# Autodesk Inventor assembly: SHOT_1_002_ShooterAssembly
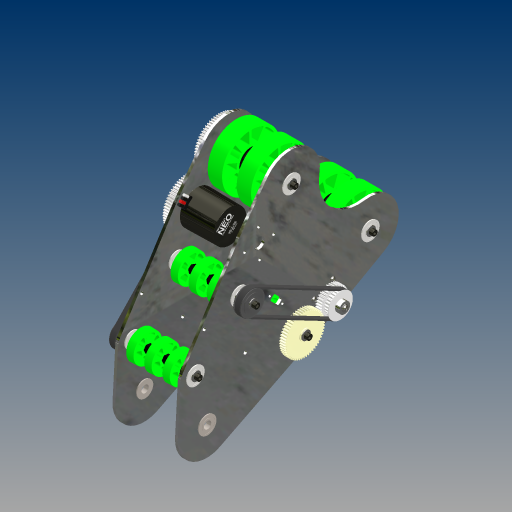
[picture p0: Inventor's stored thumbnail of the model, 512x512]
Saved by Autodesk Inventor 2024.3 (Build 283343000, 343)
## iProperties
Created: 2024-08-07
Part Number: SHOT_1_002_ShooterAssembly
Document SubType Name: Assembly
Designer: Kenji
Mass: 1474.99 g
Surface Area: 3908.93 cm^2
Volume: 710.058 cm^3
Density: 2.07728 g/cm^3
Author: Kenji
## Documents named in this file (27)
- C:\Users\Kenji\Documents\GitHub\1622-2024-Summer-CAD-A-Thon\Shooter\SHOT_1_002_ShooterAssembly.iam
- C:\Users\Kenji\Documents\GitHub\1622-2024-Summer-CAD-A-Thon\Shooter\SHOT_1_001_ShooterPlate.ipt
- C:\Users\Kenji\Documents\GitHub\1622-2024-Summer-CAD-A-Thon\COTS Library\Motion\Wheels\Compliant Wheels\4in compliant wheels\0.500in hex bore\COTS_am-3462_4indiameter_0.500inhexbore_durometer35A_CompliantWheel.ipt
- C:\Users\Kenji\Documents\GitHub\1622-2024-Summer-CAD-A-Thon\COTS Library\Motion\Bearings\COTS_WCP-0783_1.125ODHexBearing.ipt
- C:\Users\Kenji\Documents\GitHub\1622-2024-Summer-CAD-A-Thon\COTS Library\Motion\Bearings\COTS_WCP-0781_0.5ODCircularFlangedBearing.ipt
- C:\Users\Kenji\Documents\GitHub\1622-2024-Summer-CAD-A-Thon\COTS Library\Motors\COTS_REV-21-1650-V1.1_Neo1.1.ipt
- C:\Users\Kenji\Documents\GitHub\1622-2024-Summer-CAD-A-Thon\COTS Library\Motion\Wheels\Compliant Wheels\2in compliant wheels\0.500in hex bore\COTS_am-3462_2indiameter_0.500inhexbore_durometer35A_CompliantWheel.ipt
- C:\Users\Kenji\Documents\GitHub\1622-2024-Summer-CAD-A-Thon\COTS Library\Fasteners\Bolts\Button-Head\10-32\COTS_92949A265_1-2in long Stainless Steel Button Head Screw.ipt
- C:\Users\Kenji\Documents\GitHub\1622-2024-Summer-CAD-A-Thon\COTS Library\Motion\Pulleys\HTD5M\10mm Wide\COTS_HTD5M10mm24T_WCP-0564.ipt
- C:\Users\Kenji\Documents\GitHub\1622-2024-Summer-CAD-A-Thon\COTS Library\Adapters\COTS_REV-21-1879_8mmKeyTo0.5Hex.ipt
- C:\Users\Kenji\Documents\GitHub\1622-2024-Summer-CAD-A-Thon\COTS Library\Motion\Gears\20DP gears\Aluminum\COTS_WCP-0171_66T.ipt
- C:\Users\Kenji\Documents\GitHub\1622-2024-Summer-CAD-A-Thon\Shooter\SHOT_1_004_66TGear-24TPulley.ipt
- C:\Users\Kenji\Documents\GitHub\1622-2024-Summer-CAD-A-Thon\COTS Library\Motion\Gears\20DP gears\Aluminum\COTS_WCP-0717_54T.ipt
- C:\Users\Kenji\Documents\GitHub\1622-2024-Summer-CAD-A-Thon\Shooter\SHOT_1_005_36TGear-24TPulley.ipt
- C:\Users\Kenji\Documents\GitHub\1622-2024-Summer-CAD-A-Thon\Shooter\SHOT_1_014_Belt3.ipt
- C:\Users\Kenji\Documents\GitHub\1622-2024-Summer-CAD-A-Thon\Shooter\SHOT_1_013_Belt2.ipt
- C:\Users\Kenji\Documents\GitHub\1622-2024-Summer-CAD-A-Thon\Shooter\SHOT_1_012_Belt1.ipt
- C:\Users\Kenji\Documents\GitHub\1622-2024-Summer-CAD-A-Thon\Shooter\SHOT_1_010_Spacer1.ipt
- C:\Users\Kenji\Documents\GitHub\1622-2024-Summer-CAD-A-Thon\Shooter\SHOT_1_011_Spacer2.ipt
- C:\Users\Kenji\Documents\GitHub\1622-2024-Summer-CAD-A-Thon\Shooter\SHOT_1_006_HexShaft1.ipt
- C:\Users\Kenji\Documents\GitHub\1622-2024-Summer-CAD-A-Thon\Shooter\SHOT_1_007_HexShaft2.ipt
- C:\Users\Kenji\Documents\GitHub\1622-2024-Summer-CAD-A-Thon\Shooter\SHOT_1_008_HexShaft3.ipt
- C:\Users\Kenji\Documents\GitHub\1622-2024-Summer-CAD-A-Thon\Shooter\SHOT_1_009_HexShaft4.ipt
- C:\Users\Kenji\Documents\GitHub\1622-2024-Summer-CAD-A-Thon\COTS Library\Fasteners\Bolts\Socket-Head\0.25-20\COTS_91251A539_Black-Oxide Alloy Steel Socket Head Screw (1).ipt
- C:\Users\Kenji\Documents\GitHub\1622-2024-Summer-CAD-A-Thon\COTS Library\Fasteners\Washers\COTS_90107A029_316 Stainless Steel Washer.ipt
- C:\Users\Kenji\Documents\GitHub\1622-2024-Summer-CAD-A-Thon\COTS Library\Fasteners\Bolts\Button-Head\10-32\COTS_92949A267_18-8 Stainless Steel Button Head Hex Drive Screw (1).ipt
- C:\Users\Kenji\Documents\GitHub\1622-2024-Summer-CAD-A-Thon\COTS Library\Fasteners\Washers\COTS_91860A047_Size10Washer.ipt
## Components (83 placed, 26 different names)
1. SHOT_1_001_ShooterPlate:1 — Mate:140, Mate:141, Mate:142, Mate:143, Mate:144, Mate:148, Mate:150, Mate:151, Mate:152, Mate:153, Mate:155, Mate:160, Mate:161, Mate:163, Mate:164, Mate:165, Mate:166, Mate:167, Mate:168, Mate:169, Mate:170, Mate:171, Mate:172
2. SHOT_1_001_ShooterPlate:2 — Mate:140, Mate:141, Mate:145, Mate:147, Mate:149, Mate:156, Mate:157, Mate:158, Mate:159, Mate:173, Mate:174, Mate:175, Mate:176, Mate:177, Mate:178, Mate:179, Mate:180, Mate:181, Mate:183, Mate:192
3. COTS_WCP-0783_1.125ODHexBearing:1 — Mate:139, Flush:5, Mate:156, Mate:184, Mate:246
4. COTS_WCP-0783_1.125ODHexBearing:2 — Mate:146, Mate:147, Mate:149, Mate:193
5. COTS_WCP-0783_1.125ODHexBearing:3 — Mate:36, Mate:102, Flush:5, Mate:251
6. COTS_WCP-0783_1.125ODHexBearing:5 — Mate:50, Mate:136, Mate:155, Mate:244
7. COTS_WCP-0783_1.125ODHexBearing:9 — Mate:102, Flush:4, Mate:150, Mate:152, Mate:186, Mate:187
8. COTS_WCP-0783_1.125ODHexBearing:10 — Mate:31, Mate:104, Flush:4, Mate:151, Mate:188, Mate:213
9. COTS_WCP-0783_1.125ODHexBearing:11 — Mate:49, Mate:52, Mate:143, Mate:144, Mate:196, Mate:197
10. COTS_WCP-0783_1.125ODHexBearing:12 — Mate:154, Mate:157, Mate:189, Mate:190
11. COTS_WCP-0781_0.5ODCircularFlangedBearing:1 — Mate:138, Mate:158, Mate:159
12. COTS_WCP-0781_0.5ODCircularFlangedBearing:2 — Mate:138, Mate:160
13. COTS_REV-21-1650-V1.1_Neo1.1:1 — Mate:133, Mate:161, Mate:163, Mate:185, Mate:256, Mate:260, Mate:261, Mate:266
14. COTS_92949A265_1-2in long Stainless Steel Button Head Screw:1 — Mate:165, Mate:168, Mate:185
15. COTS_92949A265_1-2in long Stainless Steel Button Head Screw:2 — Mate:167, Mate:170
16. COTS_92949A265_1-2in long Stainless Steel Button Head Screw:3 — Mate:166, Mate:169
17. COTS_92949A265_1-2in long Stainless Steel Button Head Screw:4 — Mate:164, Mate:171
18. COTS_WCP-0783_1.125ODHexBearing:13 — Mate:135, Mate:148, Mate:194, Mate:195
19. COTS_WCP-0783_1.125ODHexBearing:14 — Mate:134, Mate:145, Mate:253
20. COTS_REV-21-1650-V1.1_Neo1.1:2 — Mate:123, Mate:124, Mate:173, Mate:182, Mate:183, Mate:191, Mate:258, Mate:268
21. COTS_REV-21-1879_8mmKeyTo0.5Hex:1 — Mate:123, Mate:124
22. COTS_92949A265_1-2in long Stainless Steel Button Head Screw:5 — Mate:176, Mate:178, Mate:182
23. COTS_92949A265_1-2in long Stainless Steel Button Head Screw:6 — Mate:174, Mate:181
24. COTS_92949A265_1-2in long Stainless Steel Button Head Screw:7 — Mate:175, Mate:180
25. COTS_92949A265_1-2in long Stainless Steel Button Head Screw:8 — Mate:177, Mate:179
26. SHOT_1_004_66TGear-24TPulley:1 — Mate:133, Mate:172, Flush:6, Mate:198, Mate:257
27. COTS_WCP-0171_66T:1 — Mate:186, Mate:187, Mate:206, Flush:8, Mate:241
28. COTS_HTD5M10mm24T_WCP-0564:1 — Mate:188, Flush:6, Mate:199, Mate:200, Mate:207, Flush:9, Mate:214, Mate:240
29. COTS_WCP-0717_54T:1 — Mate:189, Mate:190, Mate:208, Flush:10, Mate:254
30. SHOT_1_005_36TGear-24TPulley:1 — Mate:191, Mate:192, Flush:7, Mate:201, Mate:203, Mate:259
31. COTS_HTD5M10mm24T_WCP-0564:2 — Mate:193, Flush:7, Mate:202, Mate:212, Mate:252
32. COTS_HTD5M10mm24T_WCP-0564:3 — Mate:194, Mate:195, Mate:204, Mate:209, Flush:11, Mate:242
33. COTS_HTD5M10mm24T_WCP-0564:4 — Mate:196, Mate:197, Mate:205, Mate:210, Flush:12, Mate:243, Mate:255
34. SHOT_1_014_Belt3:1 — Mate:204, Mate:205, Mate:255
35. SHOT_1_013_Belt2:1 — Mate:201, Mate:202, Mate:203
36. SHOT_1_012_Belt1:1 — Mate:198, Mate:199, Mate:200
37. SHOT_1_010_Spacer1:1 — Mate:213, Mate:214
38. SHOT_1_010_Spacer1:2 — Mate:211, Mate:212
39. SHOT_1_006_HexShaft1:1 — Mate:206, Flush:8, Mate:235, Mate:247
40. SHOT_1_007_HexShaft2:1 — Mate:207, Flush:9, Mate:238, Mate:245
41. SHOT_1_008_HexShaft3:1 — Mate:209, Flush:11, Mate:211, Mate:236, Mate:250
42. SHOT_1_009_HexShaft4:1 — Mate:210, Flush:12, Mate:237, Mate:248
43. SHOT_1_006_HexShaft1:2 — Mate:208, Flush:10, Mate:239, Mate:249
44. COTS_91251A539_Black-Oxide Alloy Steel Socket Head Screw (1):1 — Mate:219, Mate:233, Mate:239
45. COTS_91251A539_Black-Oxide Alloy Steel Socket Head Screw (1):2 — Mate:220, Mate:230, Mate:238
46. COTS_91251A539_Black-Oxide Alloy Steel Socket Head Screw (1):3 — Mate:222, Mate:229, Mate:249
47. COTS_91251A539_Black-Oxide Alloy Steel Socket Head Screw (1):4 — Mate:217, Mate:232, Mate:247
48. COTS_91251A539_Black-Oxide Alloy Steel Socket Head Screw (1):5 — Mate:218, Mate:234, Mate:235
49. COTS_91251A539_Black-Oxide Alloy Steel Socket Head Screw (1):6 — Mate:221, Mate:226, Mate:236
50. COTS_91251A539_Black-Oxide Alloy Steel Socket Head Screw (1):7 — Mate:224, Mate:225, Mate:237
51. COTS_91251A539_Black-Oxide Alloy Steel Socket Head Screw (1):8 — Mate:223, Mate:227, Mate:250
52. COTS_91251A539_Black-Oxide Alloy Steel Socket Head Screw (1):9 — Mate:216, Mate:228, Mate:248
53. COTS_91251A539_Black-Oxide Alloy Steel Socket Head Screw (1):10 — Mate:215, Mate:231, Mate:245
54. COTS_90107A029_316 Stainless Steel Washer:1 — Mate:218, Mate:234, Mate:241
55. COTS_90107A029_316 Stainless Steel Washer:2 — Mate:220, Mate:230, Mate:240
56. COTS_90107A029_316 Stainless Steel Washer:3 — Mate:221, Mate:226, Mate:242
57. COTS_90107A029_316 Stainless Steel Washer:4 — Mate:219, Mate:233, Mate:244
58. COTS_90107A029_316 Stainless Steel Washer:5 — Mate:222, Mate:229, Mate:254
59. COTS_90107A029_316 Stainless Steel Washer:6 — Mate:223, Mate:227, Mate:252
60. COTS_90107A029_316 Stainless Steel Washer:7 — Mate:224, Mate:225, Mate:243
61. COTS_90107A029_316 Stainless Steel Washer:8 — Mate:217, Mate:232, Mate:251
62. COTS_90107A029_316 Stainless Steel Washer:9 — Mate:215, Mate:231, Mate:246
63. COTS_90107A029_316 Stainless Steel Washer:10 — Mate:216, Mate:228, Mate:253
64. SHOT_1_011_Spacer2:1 — Mate:256, Mate:257, Mate:267
65. SHOT_1_011_Spacer2:2 — Mate:258, Mate:259, Mate:269
66. COTS_REV-21-1879_8mmKeyTo0.5Hex:2 — Mate:260, Mate:261
67. COTS_92949A267_18-8 Stainless Steel Button Head Hex Drive Screw (1):1 — Mate:263, Mate:265, Mate:266
68. COTS_92949A267_18-8 Stainless Steel Button Head Hex Drive Screw (1):2 — Mate:262, Mate:264, Mate:268
69. COTS_91860A047_Size10Washer:1 — Mate:262, Mate:264, Mate:269
70. COTS_91860A047_Size10Washer:2 — Mate:263, Mate:265, Mate:267
71. COTS_am-3462_4indiameter_0.500inhexbore_durometer35A_CompliantWheel:4 — Mate:36, Flush:3
72. COTS_am-3462_4indiameter_0.500inhexbore_durometer35A_CompliantWheel:1 — Mate:31, Flush:3, Mate:104
73. COTS_am-3462_4indiameter_0.500inhexbore_durometer35A_CompliantWheel:5
74. COTS_am-3462_4indiameter_0.500inhexbore_durometer35A_CompliantWheel:6 — Mate:139, Mate:184
75. COTS_am-3462_2indiameter_0.500inhexbore_durometer35A_CompliantWheel:2 — Mate:49, Flush:1, Mate:52
76. COTS_am-3462_2indiameter_0.500inhexbore_durometer35A_CompliantWheel:6 — Flush:2, Mate:135
77. COTS_am-3462_2indiameter_0.500inhexbore_durometer35A_CompliantWheel:1 — Mate:50, Flush:1, Flush:2, Mate:136
78. COTS_am-3462_2indiameter_0.500inhexbore_durometer35A_CompliantWheel:7 — Mate:142
79. COTS_am-3462_2indiameter_0.500inhexbore_durometer35A_CompliantWheel:8
80. COTS_am-3462_2indiameter_0.500inhexbore_durometer35A_CompliantWheel:9
81. COTS_am-3462_2indiameter_0.500inhexbore_durometer35A_CompliantWheel:10 — Mate:134
82. COTS_am-3462_2indiameter_0.500inhexbore_durometer35A_CompliantWheel:11 — Mate:146
83. COTS_am-3462_2indiameter_0.500inhexbore_durometer35A_CompliantWheel:12 — Mate:153, Mate:154
## Component patterns: (2 elements, first: COTS_am-3462_4indiameter_0.500inhexbore_durometer35A_CompliantWheel:4 + COTS_am-3462_4indiameter_0.500inhexbore_durometer35A_CompliantWheel:1), (3 elements, first: COTS_am-3462_2indiameter_0.500inhexbore_durometer35A_CompliantWheel:2 + COTS_am-3462_2indiameter_0.500inhexbore_durometer35A_CompliantWheel:6 + COTS_am-3462_2indiameter_0.500inhexbore_durometer35A_CompliantWheel:1)
## Relationships (156: Mate 144, Flush 12)
- Mate:31: COTS_WCP-0783_1.125ODHexBearing:10 ↔ COTS_am-3462_4indiameter_0.500inhexbore_durometer35A_CompliantWheel:1
- Mate:36: COTS_WCP-0783_1.125ODHexBearing:3 ↔ COTS_am-3462_4indiameter_0.500inhexbore_durometer35A_CompliantWheel:4
- Mate:49: COTS_WCP-0783_1.125ODHexBearing:11 ↔ COTS_am-3462_2indiameter_0.500inhexbore_durometer35A_CompliantWheel:2
- Mate:50: COTS_WCP-0783_1.125ODHexBearing:5 ↔ COTS_am-3462_2indiameter_0.500inhexbore_durometer35A_CompliantWheel:1
- Flush:1: COTS_am-3462_2indiameter_0.500inhexbore_durometer35A_CompliantWheel:2 ↔ COTS_am-3462_2indiameter_0.500inhexbore_durometer35A_CompliantWheel:1
- Flush:2: COTS_am-3462_2indiameter_0.500inhexbore_durometer35A_CompliantWheel:6 ↔ COTS_am-3462_2indiameter_0.500inhexbore_durometer35A_CompliantWheel:1
- Mate:52 (12.7 mm): COTS_WCP-0783_1.125ODHexBearing:11 ↔ COTS_am-3462_2indiameter_0.500inhexbore_durometer35A_CompliantWheel:2
- Mate:102: COTS_WCP-0783_1.125ODHexBearing:3 ↔ COTS_WCP-0783_1.125ODHexBearing:9
- Flush:3: COTS_am-3462_4indiameter_0.500inhexbore_durometer35A_CompliantWheel:4 ↔ COTS_am-3462_4indiameter_0.500inhexbore_durometer35A_CompliantWheel:1
- Mate:104 (12.7 mm): COTS_WCP-0783_1.125ODHexBearing:10 ↔ COTS_am-3462_4indiameter_0.500inhexbore_durometer35A_CompliantWheel:1
- Mate:123: COTS_REV-21-1650-V1.1_Neo1.1:2 ↔ COTS_REV-21-1879_8mmKeyTo0.5Hex:1
- Mate:124: COTS_REV-21-1650-V1.1_Neo1.1:2 ↔ COTS_REV-21-1879_8mmKeyTo0.5Hex:1
- Mate:133: COTS_REV-21-1650-V1.1_Neo1.1:1 ↔ SHOT_1_004_66TGear-24TPulley:1
- Mate:134: COTS_WCP-0783_1.125ODHexBearing:14 ↔ COTS_am-3462_2indiameter_0.500inhexbore_durometer35A_CompliantWheel:10
- Mate:135: COTS_WCP-0783_1.125ODHexBearing:13 ↔ COTS_am-3462_2indiameter_0.500inhexbore_durometer35A_CompliantWheel:6
- Mate:136: COTS_WCP-0783_1.125ODHexBearing:5 ↔ COTS_am-3462_2indiameter_0.500inhexbore_durometer35A_CompliantWheel:1
- Mate:138: COTS_WCP-0781_0.5ODCircularFlangedBearing:1 ↔ COTS_WCP-0781_0.5ODCircularFlangedBearing:2
- Mate:139: COTS_WCP-0783_1.125ODHexBearing:1 ↔ COTS_am-3462_4indiameter_0.500inhexbore_durometer35A_CompliantWheel:6
- Flush:4: COTS_WCP-0783_1.125ODHexBearing:9 ↔ COTS_WCP-0783_1.125ODHexBearing:10
- Flush:5: COTS_WCP-0783_1.125ODHexBearing:1 ↔ COTS_WCP-0783_1.125ODHexBearing:3
- Mate:140: SHOT_1_001_ShooterPlate:1 ↔ SHOT_1_001_ShooterPlate:2
- Mate:141: SHOT_1_001_ShooterPlate:1 ↔ SHOT_1_001_ShooterPlate:2
- Mate:142: SHOT_1_001_ShooterPlate:1 ↔ COTS_am-3462_2indiameter_0.500inhexbore_durometer35A_CompliantWheel:7
- Mate:143: SHOT_1_001_ShooterPlate:1 ↔ COTS_WCP-0783_1.125ODHexBearing:11
- Mate:144: SHOT_1_001_ShooterPlate:1 ↔ COTS_WCP-0783_1.125ODHexBearing:11
- Mate:145: SHOT_1_001_ShooterPlate:2 ↔ COTS_WCP-0783_1.125ODHexBearing:14
- Mate:146: COTS_WCP-0783_1.125ODHexBearing:2 ↔ COTS_am-3462_2indiameter_0.500inhexbore_durometer35A_CompliantWheel:11
- Mate:147: SHOT_1_001_ShooterPlate:2 ↔ COTS_WCP-0783_1.125ODHexBearing:2
- Mate:148: SHOT_1_001_ShooterPlate:1 ↔ COTS_WCP-0783_1.125ODHexBearing:13
- Mate:149: SHOT_1_001_ShooterPlate:2 ↔ COTS_WCP-0783_1.125ODHexBearing:2
- Mate:150: SHOT_1_001_ShooterPlate:1 ↔ COTS_WCP-0783_1.125ODHexBearing:9
- Mate:151: SHOT_1_001_ShooterPlate:1 ↔ COTS_WCP-0783_1.125ODHexBearing:10
- Mate:152: SHOT_1_001_ShooterPlate:1 ↔ COTS_WCP-0783_1.125ODHexBearing:9
- Mate:153: SHOT_1_001_ShooterPlate:1 ↔ COTS_am-3462_2indiameter_0.500inhexbore_durometer35A_CompliantWheel:12
- Mate:154: COTS_WCP-0783_1.125ODHexBearing:12 ↔ COTS_am-3462_2indiameter_0.500inhexbore_durometer35A_CompliantWheel:12
- Mate:155: SHOT_1_001_ShooterPlate:1 ↔ COTS_WCP-0783_1.125ODHexBearing:5
- Mate:156: SHOT_1_001_ShooterPlate:2 ↔ COTS_WCP-0783_1.125ODHexBearing:1
- Mate:157: SHOT_1_001_ShooterPlate:2 ↔ COTS_WCP-0783_1.125ODHexBearing:12
- Mate:158: SHOT_1_001_ShooterPlate:2 ↔ COTS_WCP-0781_0.5ODCircularFlangedBearing:1
- Mate:159: SHOT_1_001_ShooterPlate:2 ↔ COTS_WCP-0781_0.5ODCircularFlangedBearing:1
- Mate:160: SHOT_1_001_ShooterPlate:1 ↔ COTS_WCP-0781_0.5ODCircularFlangedBearing:2
- Mate:161: SHOT_1_001_ShooterPlate:1 ↔ COTS_REV-21-1650-V1.1_Neo1.1:1
- Mate:163: SHOT_1_001_ShooterPlate:1 ↔ COTS_REV-21-1650-V1.1_Neo1.1:1
- Mate:164: SHOT_1_001_ShooterPlate:1 ↔ COTS_92949A265_1-2in long Stainless Steel Button Head Screw:4
- Mate:165: SHOT_1_001_ShooterPlate:1 ↔ COTS_92949A265_1-2in long Stainless Steel Button Head Screw:1
- Mate:166: SHOT_1_001_ShooterPlate:1 ↔ COTS_92949A265_1-2in long Stainless Steel Button Head Screw:3
- Mate:167: SHOT_1_001_ShooterPlate:1 ↔ COTS_92949A265_1-2in long Stainless Steel Button Head Screw:2
- Mate:168: SHOT_1_001_ShooterPlate:1 ↔ COTS_92949A265_1-2in long Stainless Steel Button Head Screw:1
- Mate:169: SHOT_1_001_ShooterPlate:1 ↔ COTS_92949A265_1-2in long Stainless Steel Button Head Screw:3
- Mate:170: SHOT_1_001_ShooterPlate:1 ↔ COTS_92949A265_1-2in long Stainless Steel Button Head Screw:2
- Mate:171: SHOT_1_001_ShooterPlate:1 ↔ COTS_92949A265_1-2in long Stainless Steel Button Head Screw:4
- Mate:172: SHOT_1_001_ShooterPlate:1 ↔ SHOT_1_004_66TGear-24TPulley:1
- Mate:173: SHOT_1_001_ShooterPlate:2 ↔ COTS_REV-21-1650-V1.1_Neo1.1:2
- Mate:174: SHOT_1_001_ShooterPlate:2 ↔ COTS_92949A265_1-2in long Stainless Steel Button Head Screw:6
- Mate:175: SHOT_1_001_ShooterPlate:2 ↔ COTS_92949A265_1-2in long Stainless Steel Button Head Screw:7
- Mate:176: SHOT_1_001_ShooterPlate:2 ↔ COTS_92949A265_1-2in long Stainless Steel Button Head Screw:5
- Mate:177: SHOT_1_001_ShooterPlate:2 ↔ COTS_92949A265_1-2in long Stainless Steel Button Head Screw:8
- Mate:178: SHOT_1_001_ShooterPlate:2 ↔ COTS_92949A265_1-2in long Stainless Steel Button Head Screw:5
- Mate:179: SHOT_1_001_ShooterPlate:2 ↔ COTS_92949A265_1-2in long Stainless Steel Button Head Screw:8
- Mate:180: SHOT_1_001_ShooterPlate:2 ↔ COTS_92949A265_1-2in long Stainless Steel Button Head Screw:7
- Mate:181: SHOT_1_001_ShooterPlate:2 ↔ COTS_92949A265_1-2in long Stainless Steel Button Head Screw:6
- Mate:182: COTS_REV-21-1650-V1.1_Neo1.1:2 ↔ COTS_92949A265_1-2in long Stainless Steel Button Head Screw:5
- Mate:183: SHOT_1_001_ShooterPlate:2 ↔ COTS_REV-21-1650-V1.1_Neo1.1:2
- Mate:184 (12.7 mm): COTS_WCP-0783_1.125ODHexBearing:1 ↔ COTS_am-3462_4indiameter_0.500inhexbore_durometer35A_CompliantWheel:6
- Mate:185: COTS_REV-21-1650-V1.1_Neo1.1:1 ↔ COTS_92949A265_1-2in long Stainless Steel Button Head Screw:1
- Mate:186: COTS_WCP-0783_1.125ODHexBearing:9 ↔ COTS_WCP-0171_66T:1
- Mate:187: COTS_WCP-0783_1.125ODHexBearing:9 ↔ COTS_WCP-0171_66T:1
- Mate:188: COTS_WCP-0783_1.125ODHexBearing:10 ↔ COTS_HTD5M10mm24T_WCP-0564:1
- Flush:6: SHOT_1_004_66TGear-24TPulley:1 ↔ COTS_HTD5M10mm24T_WCP-0564:1
- Mate:189: COTS_WCP-0783_1.125ODHexBearing:12 ↔ COTS_WCP-0717_54T:1
- Mate:190: COTS_WCP-0783_1.125ODHexBearing:12 ↔ COTS_WCP-0717_54T:1
- Mate:191: COTS_REV-21-1650-V1.1_Neo1.1:2 ↔ SHOT_1_005_36TGear-24TPulley:1
- Mate:192: SHOT_1_001_ShooterPlate:2 ↔ SHOT_1_005_36TGear-24TPulley:1
- Mate:193: COTS_WCP-0783_1.125ODHexBearing:2 ↔ COTS_HTD5M10mm24T_WCP-0564:2
- Flush:7: SHOT_1_005_36TGear-24TPulley:1 ↔ COTS_HTD5M10mm24T_WCP-0564:2
- Mate:194: COTS_WCP-0783_1.125ODHexBearing:13 ↔ COTS_HTD5M10mm24T_WCP-0564:3
- Mate:195: COTS_WCP-0783_1.125ODHexBearing:13 ↔ COTS_HTD5M10mm24T_WCP-0564:3
- Mate:196: COTS_WCP-0783_1.125ODHexBearing:11 ↔ COTS_HTD5M10mm24T_WCP-0564:4
- Mate:197: COTS_WCP-0783_1.125ODHexBearing:11 ↔ COTS_HTD5M10mm24T_WCP-0564:4
- Mate:198: SHOT_1_004_66TGear-24TPulley:1 ↔ SHOT_1_012_Belt1:1
- Mate:199: COTS_HTD5M10mm24T_WCP-0564:1 ↔ SHOT_1_012_Belt1:1
- Mate:200: COTS_HTD5M10mm24T_WCP-0564:1 ↔ SHOT_1_012_Belt1:1
- Mate:201: SHOT_1_005_36TGear-24TPulley:1 ↔ SHOT_1_013_Belt2:1
- Mate:202: COTS_HTD5M10mm24T_WCP-0564:2 ↔ SHOT_1_013_Belt2:1
- Mate:203: SHOT_1_005_36TGear-24TPulley:1 ↔ SHOT_1_013_Belt2:1
- Mate:204: COTS_HTD5M10mm24T_WCP-0564:3 ↔ SHOT_1_014_Belt3:1
- Mate:205: COTS_HTD5M10mm24T_WCP-0564:4 ↔ SHOT_1_014_Belt3:1
- Mate:206: COTS_WCP-0171_66T:1 ↔ SHOT_1_006_HexShaft1:1
- Flush:8: COTS_WCP-0171_66T:1 ↔ SHOT_1_006_HexShaft1:1
- Mate:207: COTS_HTD5M10mm24T_WCP-0564:1 ↔ SHOT_1_007_HexShaft2:1
- Flush:9: COTS_HTD5M10mm24T_WCP-0564:1 ↔ SHOT_1_007_HexShaft2:1
- Mate:208: COTS_WCP-0717_54T:1 ↔ SHOT_1_006_HexShaft1:2
- Flush:10: COTS_WCP-0717_54T:1 ↔ SHOT_1_006_HexShaft1:2
- Mate:209: COTS_HTD5M10mm24T_WCP-0564:3 ↔ SHOT_1_008_HexShaft3:1
- Flush:11: COTS_HTD5M10mm24T_WCP-0564:3 ↔ SHOT_1_008_HexShaft3:1
- Mate:210: COTS_HTD5M10mm24T_WCP-0564:4 ↔ SHOT_1_009_HexShaft4:1
- Flush:12: COTS_HTD5M10mm24T_WCP-0564:4 ↔ SHOT_1_009_HexShaft4:1
- Mate:211: SHOT_1_010_Spacer1:2 ↔ SHOT_1_008_HexShaft3:1
- Mate:212: COTS_HTD5M10mm24T_WCP-0564:2 ↔ SHOT_1_010_Spacer1:2
- Mate:213: COTS_WCP-0783_1.125ODHexBearing:10 ↔ SHOT_1_010_Spacer1:1
- Mate:214: COTS_HTD5M10mm24T_WCP-0564:1 ↔ SHOT_1_010_Spacer1:1
- Mate:215: COTS_91251A539_Black-Oxide Alloy Steel Socket Head Screw (1):10 ↔ COTS_90107A029_316 Stainless Steel Washer:9
- Mate:216: COTS_91251A539_Black-Oxide Alloy Steel Socket Head Screw (1):9 ↔ COTS_90107A029_316 Stainless Steel Washer:10
- Mate:217: COTS_91251A539_Black-Oxide Alloy Steel Socket Head Screw (1):4 ↔ COTS_90107A029_316 Stainless Steel Washer:8
- Mate:218: COTS_91251A539_Black-Oxide Alloy Steel Socket Head Screw (1):5 ↔ COTS_90107A029_316 Stainless Steel Washer:1
- Mate:219: COTS_91251A539_Black-Oxide Alloy Steel Socket Head Screw (1):1 ↔ COTS_90107A029_316 Stainless Steel Washer:4
- Mate:220: COTS_91251A539_Black-Oxide Alloy Steel Socket Head Screw (1):2 ↔ COTS_90107A029_316 Stainless Steel Washer:2
- Mate:221: COTS_91251A539_Black-Oxide Alloy Steel Socket Head Screw (1):6 ↔ COTS_90107A029_316 Stainless Steel Washer:3
- Mate:222: COTS_91251A539_Black-Oxide Alloy Steel Socket Head Screw (1):3 ↔ COTS_90107A029_316 Stainless Steel Washer:5
- Mate:223: COTS_91251A539_Black-Oxide Alloy Steel Socket Head Screw (1):8 ↔ COTS_90107A029_316 Stainless Steel Washer:6
- Mate:224: COTS_91251A539_Black-Oxide Alloy Steel Socket Head Screw (1):7 ↔ COTS_90107A029_316 Stainless Steel Washer:7
- Mate:225: COTS_91251A539_Black-Oxide Alloy Steel Socket Head Screw (1):7 ↔ COTS_90107A029_316 Stainless Steel Washer:7
- Mate:226: COTS_91251A539_Black-Oxide Alloy Steel Socket Head Screw (1):6 ↔ COTS_90107A029_316 Stainless Steel Washer:3
- Mate:227: COTS_91251A539_Black-Oxide Alloy Steel Socket Head Screw (1):8 ↔ COTS_90107A029_316 Stainless Steel Washer:6
- Mate:228: COTS_91251A539_Black-Oxide Alloy Steel Socket Head Screw (1):9 ↔ COTS_90107A029_316 Stainless Steel Washer:10
- Mate:229: COTS_91251A539_Black-Oxide Alloy Steel Socket Head Screw (1):3 ↔ COTS_90107A029_316 Stainless Steel Washer:5
- Mate:230: COTS_91251A539_Black-Oxide Alloy Steel Socket Head Screw (1):2 ↔ COTS_90107A029_316 Stainless Steel Washer:2
- Mate:231: COTS_91251A539_Black-Oxide Alloy Steel Socket Head Screw (1):10 ↔ COTS_90107A029_316 Stainless Steel Washer:9
- Mate:232: COTS_91251A539_Black-Oxide Alloy Steel Socket Head Screw (1):4 ↔ COTS_90107A029_316 Stainless Steel Washer:8
- Mate:233: COTS_91251A539_Black-Oxide Alloy Steel Socket Head Screw (1):1 ↔ COTS_90107A029_316 Stainless Steel Washer:4
- Mate:234: COTS_91251A539_Black-Oxide Alloy Steel Socket Head Screw (1):5 ↔ COTS_90107A029_316 Stainless Steel Washer:1
- Mate:235: SHOT_1_006_HexShaft1:1 ↔ COTS_91251A539_Black-Oxide Alloy Steel Socket Head Screw (1):5
- Mate:236: SHOT_1_008_HexShaft3:1 ↔ COTS_91251A539_Black-Oxide Alloy Steel Socket Head Screw (1):6
- Mate:237: SHOT_1_009_HexShaft4:1 ↔ COTS_91251A539_Black-Oxide Alloy Steel Socket Head Screw (1):7
- Mate:238: SHOT_1_007_HexShaft2:1 ↔ COTS_91251A539_Black-Oxide Alloy Steel Socket Head Screw (1):2
- Mate:239: SHOT_1_006_HexShaft1:2 ↔ COTS_91251A539_Black-Oxide Alloy Steel Socket Head Screw (1):1
- Mate:240: COTS_HTD5M10mm24T_WCP-0564:1 ↔ COTS_90107A029_316 Stainless Steel Washer:2
- Mate:241: COTS_WCP-0171_66T:1 ↔ COTS_90107A029_316 Stainless Steel Washer:1
- Mate:242: COTS_HTD5M10mm24T_WCP-0564:3 ↔ COTS_90107A029_316 Stainless Steel Washer:3
- Mate:243: COTS_HTD5M10mm24T_WCP-0564:4 ↔ COTS_90107A029_316 Stainless Steel Washer:7
- Mate:244: COTS_WCP-0783_1.125ODHexBearing:5 ↔ COTS_90107A029_316 Stainless Steel Washer:4
- Mate:245: SHOT_1_007_HexShaft2:1 ↔ COTS_91251A539_Black-Oxide Alloy Steel Socket Head Screw (1):10
- Mate:246: COTS_WCP-0783_1.125ODHexBearing:1 ↔ COTS_90107A029_316 Stainless Steel Washer:9
- Mate:247: SHOT_1_006_HexShaft1:1 ↔ COTS_91251A539_Black-Oxide Alloy Steel Socket Head Screw (1):4
- Mate:248: SHOT_1_009_HexShaft4:1 ↔ COTS_91251A539_Black-Oxide Alloy Steel Socket Head Screw (1):9
- Mate:249: SHOT_1_006_HexShaft1:2 ↔ COTS_91251A539_Black-Oxide Alloy Steel Socket Head Screw (1):3
- Mate:250: SHOT_1_008_HexShaft3:1 ↔ COTS_91251A539_Black-Oxide Alloy Steel Socket Head Screw (1):8
- Mate:251: COTS_WCP-0783_1.125ODHexBearing:3 ↔ COTS_90107A029_316 Stainless Steel Washer:8
- Mate:252: COTS_HTD5M10mm24T_WCP-0564:2 ↔ COTS_90107A029_316 Stainless Steel Washer:6
- Mate:253: COTS_WCP-0783_1.125ODHexBearing:14 ↔ COTS_90107A029_316 Stainless Steel Washer:10
- Mate:254: COTS_WCP-0717_54T:1 ↔ COTS_90107A029_316 Stainless Steel Washer:5
- Mate:255: COTS_HTD5M10mm24T_WCP-0564:4 ↔ SHOT_1_014_Belt3:1
- Mate:256: COTS_REV-21-1650-V1.1_Neo1.1:1 ↔ SHOT_1_011_Spacer2:1
- Mate:257: SHOT_1_004_66TGear-24TPulley:1 ↔ SHOT_1_011_Spacer2:1
- Mate:258: COTS_REV-21-1650-V1.1_Neo1.1:2 ↔ SHOT_1_011_Spacer2:2
- Mate:259: SHOT_1_005_36TGear-24TPulley:1 ↔ SHOT_1_011_Spacer2:2
- Mate:260: COTS_REV-21-1650-V1.1_Neo1.1:1 ↔ COTS_REV-21-1879_8mmKeyTo0.5Hex:2
- Mate:261: COTS_REV-21-1650-V1.1_Neo1.1:1 ↔ COTS_REV-21-1879_8mmKeyTo0.5Hex:2
- Mate:262: COTS_92949A267_18-8 Stainless Steel Button Head Hex Drive Screw (1):2 ↔ COTS_91860A047_Size10Washer:1
- Mate:263: COTS_92949A267_18-8 Stainless Steel Button Head Hex Drive Screw (1):1 ↔ COTS_91860A047_Size10Washer:2
- Mate:264: COTS_92949A267_18-8 Stainless Steel Button Head Hex Drive Screw (1):2 ↔ COTS_91860A047_Size10Washer:1
- Mate:265: COTS_92949A267_18-8 Stainless Steel Button Head Hex Drive Screw (1):1 ↔ COTS_91860A047_Size10Washer:2
- Mate:266: COTS_REV-21-1650-V1.1_Neo1.1:1 ↔ COTS_92949A267_18-8 Stainless Steel Button Head Hex Drive Screw (1):1
- Mate:267: SHOT_1_011_Spacer2:1 ↔ COTS_91860A047_Size10Washer:2
- Mate:268: COTS_REV-21-1650-V1.1_Neo1.1:2 ↔ COTS_92949A267_18-8 Stainless Steel Button Head Hex Drive Screw (1):2
- Mate:269: SHOT_1_011_Spacer2:2 ↔ COTS_91860A047_Size10Washer:1
